# Autodesk Inventor assembly: Assembly2
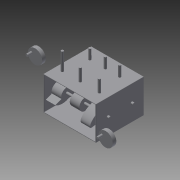
[picture p0: Inventor's stored thumbnail of the model, 180x180]
Saved by Autodesk Inventor 2014 (Build 180170000, 170)
## iProperties
Created: 2014-05-19
Part Number: Assembly2
Document SubType Name: Assembly
Designer: jyesowitz
Author: jyesowitz
## Documents named in this file (8)
- C:\Users\jyesowitz\Documents\GitHub\FinalProjectFirst\Assembly2.iam
- C:\Users\jyesowitz\Documents\GitHub\FinalProjectFirst\cam 1.ipt
- C:\Users\jyesowitz\Documents\GitHub\FinalProjectFirst\cam 2.ipt
- C:\Users\jyesowitz\Documents\GitHub\FinalProjectFirst\cam 3.ipt
- C:\Users\jyesowitz\Documents\GitHub\FinalProjectFirst\rod.ipt
- C:\Users\jyesowitz\Documents\GitHub\FinalProjectFirst\Box Base.ipt
- C:\Users\jyesowitz\Documents\GitHub\FinalProjectFirst\crank.ipt
- C:\Users\jyesowitz\Documents\GitHub\FinalProjectFirst\moving ball thing.ipt
## Components (17 placed, 7 different names)
1. cam 1:1 — Insert:3, Flush:1
2. cam 2:1 — Insert:1, Angle:1, Flush:2
3. cam 3:1 — Insert:2, Mate:3
4. rod:1 — Insert:1, Insert:2, Insert:3, Insert:7
5. cam 1:2 — Insert:5, Flush:5, Flush:6
6. cam 2:2 — Insert:6, Flush:4
7. cam 3:2 — Insert:4, Flush:3
8. rod:2 — Insert:4, Insert:5, Insert:6, Insert:8
9. Box Base:1 — Insert:7, Insert:8, Mate:1, Mate:2, Mate:4, Angle:2, Mate:5, Angle:3, Mate:6, Angle:4, Mate:7, Angle:5, Mate:8, Angle:6, Mate:9, Angle:7
10. crank:1
11. crank:2
12. moving ball thing:1 — Mate:4, Angle:2
13. moving ball thing:2 — Mate:8, Angle:6
14. moving ball thing:3 — Mate:5, Angle:3
15. moving ball thing:4 — Mate:9, Angle:7
16. moving ball thing:5 — Mate:7, Angle:5
17. moving ball thing:6 — Mate:6, Angle:4
## Relationships (30: Mate 9, Insert 8, Angle 7, Flush 6)
- Insert:1 (50.8 mm): cam 2:1 ↔ rod:1
- Insert:2 (44.45 mm): cam 3:1 ↔ rod:1
- Insert:3 (127 mm): cam 1:1 ↔ rod:1
- Insert:4 (31.75 mm): cam 3:2 ↔ rod:2
- Insert:5 (25.4 mm): cam 1:2 ↔ rod:2
- Insert:6 (133.35 mm): cam 2:2 ↔ rod:2
- Insert:7 (-12.7 mm): rod:1 ↔ Box Base:1
- Insert:8 (-12.7 mm): rod:2 ↔ Box Base:1
- Mate:1: Box Base:1
- Mate:2: Box Base:1
- Mate:3: cam 3:1
- Angle:1 (0 deg): cam 2:1
- Flush:1: cam 1:1
- Flush:2: cam 2:1
- Flush:3: cam 3:2
- Flush:4: cam 2:2
- Flush:5: cam 1:2
- Flush:6: cam 1:2
- Mate:4: Box Base:1 ↔ moving ball thing:1
- Angle:2 (0 deg): Box Base:1 ↔ moving ball thing:1
- Mate:5: Box Base:1 ↔ moving ball thing:3
- Angle:3 (0 deg): Box Base:1 ↔ moving ball thing:3
- Mate:6: Box Base:1 ↔ moving ball thing:6
- Angle:4 (0 deg): Box Base:1 ↔ moving ball thing:6
- Mate:7: Box Base:1 ↔ moving ball thing:5
- Angle:5 (0 deg): Box Base:1 ↔ moving ball thing:5
- Mate:8: Box Base:1 ↔ moving ball thing:2
- Angle:6 (0 deg): Box Base:1 ↔ moving ball thing:2
- Mate:9: Box Base:1 ↔ moving ball thing:4
- Angle:7 (0 deg): Box Base:1 ↔ moving ball thing:4
